# Autodesk Inventor assembly: Intake
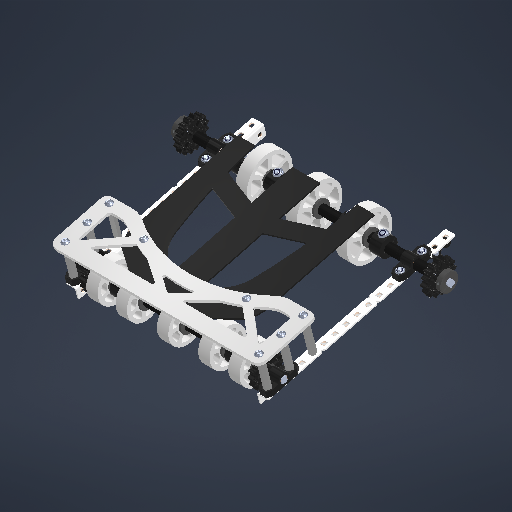
[picture p0: Inventor's stored thumbnail of the model, 512x512]
Saved by Autodesk Inventor 2025 (Build 290162000, 162)
## iProperties
Created: 2024-12-18
Part Number: Intake
Document SubType Name: Assembly
Designer: Juan
Author: Juan
## Documents named in this file (30)
- C:\Users\Juan\Documents\GitHub\ATUM-VRC-High-Stakes-CAD\Robot\Subassemblies\Intake.iam
- C:\Users\Juan\Documents\GitHub\ATUM-VRC-High-Stakes-CAD\VEX-CAD-Inventor\Motion\Shaft HS\Shaft HS\Shaft HS 9.0 in.ipt
- C:\Users\Juan\Documents\GitHub\ATUM-VRC-High-Stakes-CAD\VEX-CAD-Inventor\Motion\Shaft HS\Shaft HS.ipt
- C:\Users\Juan\Documents\GitHub\ATUM-VRC-High-Stakes-CAD\VEX-CAD-Inventor\Structure\Angle\Aluminum 1x1\Alu Angle 1x1x17.ipt
- C:\Users\Juan\Documents\GitHub\ATUM-VRC-High-Stakes-CAD\VEX-CAD-Inventor\Motion\Shaft HS\HS Pillow Bearing Block.ipt
- C:\Users\Juan\Documents\GitHub\ATUM-VRC-High-Stakes-CAD\VEX-CAD-Inventor\Motion\Sprockets\6P Sprocket\6P 16T Sprocket, No Insert.iam
- C:\Users\Juan\Documents\GitHub\ATUM-VRC-High-Stakes-CAD\VEX-CAD-Inventor\Motion\Sprockets\6P Sprocket.iam
- C:\Users\Juan\Documents\GitHub\ATUM-VRC-High-Stakes-CAD\VEX-CAD-Inventor\Structure\Hardware\Screw Steel - Star\SScrew Star Threaded .375.ipt
- C:\Users\Juan\Documents\GitHub\ATUM-VRC-High-Stakes-CAD\VEX-CAD-Inventor\Structure\Hardware\Screw Steel - Star.ipt
- C:\Users\Juan\Documents\GitHub\ATUM-VRC-High-Stakes-CAD\VEX-CAD-Inventor\Structure\Standoff\Standoff 1.50.ipt
- C:\Users\Juan\Documents\GitHub\ATUM-VRC-High-Stakes-CAD\VEX-CAD-Inventor\Structure\Standoff.ipt
- C:\Users\Juan\Documents\GitHub\ATUM-VRC-High-Stakes-CAD\VEX-CAD-Inventor\Motion\1-Post Bearing Flat Hex Retainer.ipt
- C:\Users\Juan\Documents\GitHub\ATUM-VRC-High-Stakes-CAD\VEX-CAD-Inventor\Motion\Shaft HS\Shaft HS\Shaft HS 12.0 in.ipt
- C:\Users\Juan\Documents\GitHub\ATUM-VRC-High-Stakes-CAD\VEX-CAD-Inventor\Motion\Shaft HS\HS Shaft Collar.ipt
- C:\Users\Juan\Documents\GitHub\ATUM-VRC-High-Stakes-CAD\VEX-CAD-Inventor\Motion\Shaft HS\HS Spacer\HSpacer .5000.ipt
- C:\Users\Juan\Documents\GitHub\ATUM-VRC-High-Stakes-CAD\VEX-CAD-Inventor\Motion\Shaft HS\HS Spacer.ipt
- C:\Users\Juan\Documents\GitHub\ATUM-VRC-High-Stakes-CAD\VEX-CAD-Inventor\Motion\Shaft HS\Low Profile HS Shaft Collar.ipt
- C:\Users\Juan\Documents\GitHub\ATUM-VRC-High-Stakes-CAD\VEX-CAD-Inventor\Motion\Shaft HS\HS Spacer\HSpacer .2500.ipt
- C:\Users\Juan\Documents\GitHub\ATUM-VRC-High-Stakes-CAD\Robot\Subassemblies\2.0 Flex Wheel with Insert.iam
- C:\Users\Juan\Documents\GitHub\ATUM-VRC-High-Stakes-CAD\VEX-CAD-Inventor\Structure\Hardware\Nut Thin Nylock.ipt
- C:\Users\Juan\Documents\GitHub\ATUM-VRC-High-Stakes-CAD\VEX-CAD-Inventor\Structure\Hardware\Screw Steel - Star\SScrew Star Smooth .625.ipt
- C:\Users\Juan\Documents\GitHub\ATUM-VRC-High-Stakes-CAD\VEX-CAD-Inventor\Motion\Shaft HS\HS Spacer\HSpacer .1250.ipt
- C:\Users\Juan\Documents\GitHub\ATUM-VRC-High-Stakes-CAD\VEX-CAD-Inventor\Motion\Shaft HS\HS Spacer\HSpacer .0625.ipt
- C:\Users\Juan\Documents\GitHub\ATUM-VRC-High-Stakes-CAD\VEX-CAD-Inventor\Structure\Hardware\Screw Steel - Star\SScrew Star Smooth .375.ipt
- C:\Users\Juan\Documents\GitHub\ATUM-VRC-High-Stakes-CAD\Robot\Subassemblies\1.625 Flex Wheel with Insert.iam
- C:\Users\Juan\Documents\GitHub\ATUM-VRC-High-Stakes-CAD\Protobot\Intake (Metal).ipt
- C:\Users\Juan\Documents\GitHub\ATUM-VRC-High-Stakes-CAD\VEX-CAD-Inventor\Motion\Spacers\Washer Steel\SWasher .375 OD x .062500.ipt
- C:\Users\Juan\Documents\GitHub\ATUM-VRC-High-Stakes-CAD\VEX-CAD-Inventor\Motion\Spacers\Washer Steel.ipt
- C:\Users\Juan\Documents\GitHub\ATUM-VRC-High-Stakes-CAD\VEX-CAD-Inventor\Motion\Spacers\Washer Steel\SWasher .375 OD x .015625.ipt
- C:\Users\Juan\Documents\GitHub\ATUM-VRC-High-Stakes-CAD\Protobot\Intake Hood.ipt
## Components (104 placed, 23 different names)
1. Shaft HS 9.0 in:1
2. Alu Angle 1x1x17:1 — Rigid:31, Rigid:37
3. HS Pillow Bearing Block:4
4. Alu Angle 1x1x17:2 — Rigid:32, Rigid:56
5. HS Pillow Bearing Block:1
6. HS Pillow Bearing Block:2
7. 6P 16T Sprocket, No Insert:1 [sub-assembly]
8. 6P 16T Sprocket, No Insert:2 [sub-assembly]
9. SScrew Star Threaded .375:1
10. Standoff 1.50:1 — Mate:120, Mate:122
11. Standoff 1.50:2 — Mate:121
12. Standoff 1.50:3
13. Standoff 1.50:4
14. 1-Post Bearing Flat Hex Retainer:1
15. HS Pillow Bearing Block:3
16. Shaft HS 12.0 in:2
17. 6P 16T Sprocket, No Insert:3 [sub-assembly]
18. 6P 16T Sprocket, No Insert:4 [sub-assembly]
19. HS Shaft Collar:1
20. HS Shaft Collar:2
21. HSpacer .5000:1
22. HSpacer .5000:2
23. HSpacer .5000:3
24. HSpacer .5000:4
25. Low Profile HS Shaft Collar:1
26. Low Profile HS Shaft Collar:2
27. HS Shaft Collar:3
28. HS Shaft Collar:4
29. HSpacer .2500:5
30. HSpacer .2500:6
31. 2.0 Flex Wheel with Insert:1 [sub-assembly]
32. 1-Post Bearing Flat Hex Retainer:2
33. 2.0 Flex Wheel with Insert:2 [sub-assembly]
34. 2.0 Flex Wheel with Insert:3 [sub-assembly]
35. HSpacer .5000:7
36. Nut Thin Nylock:1
37. HSpacer .5000:8
38. SScrew Star Smooth .625:2
39. SScrew Star Smooth .625:3
40. SScrew Star Smooth .625:4
41. SScrew Star Smooth .625:5
42. Nut Thin Nylock:2
43. Nut Thin Nylock:3
44. Nut Thin Nylock:4
45. HSpacer .5000:9
46. HSpacer .5000:10
47. HSpacer .1250:11
48. HSpacer .1250:12
49. HSpacer .0625:13
50. HSpacer .1250:14
51. HSpacer .1250:15
52. HSpacer .0625:16
53. HSpacer .0625:17
54. Nut Thin Nylock:5
55. Nut Thin Nylock:6
56. Nut Thin Nylock:7
57. Nut Thin Nylock:8
58. SScrew Star Smooth .375:6
59. SScrew Star Smooth .375:7
60. SScrew Star Smooth .375:8
61. SScrew Star Smooth .375:9
62. SScrew Star Smooth .375:14
63. SScrew Star Smooth .375:15
64. SScrew Star Smooth .375:16
65. SScrew Star Smooth .375:17
66. 1.625 Flex Wheel with Insert:1 [sub-assembly]
67. 1.625 Flex Wheel with Insert:2 [sub-assembly]
68. 1.625 Flex Wheel with Insert:3 [sub-assembly]
69. 1.625 Flex Wheel with Insert:4 [sub-assembly]
70. 1.625 Flex Wheel with Insert:5 [sub-assembly]
71. HSpacer .5000:18
72. HSpacer .1250:19
73. HSpacer .1250:20
74. HSpacer .5000:21
75. HSpacer .5000:22
76. HSpacer .5000:23
77. HS Shaft Collar:5
78. Nut Thin Nylock:9
79. SScrew Star Smooth .625:18
80. HS Shaft Collar:6
81. Nut Thin Nylock:10
82. SScrew Star Smooth .625:19
83. HSpacer .1250:24
84. HSpacer .1250:25
85. Intake (Metal):1 — Mate:120, Mate:121, Mate:122, Rigid:38, Rigid:39, Rigid:40, Rigid:41, Rigid:42, Rigid:43, Mate:125, Rigid:44, Rigid:48, Mate:126
86. Standoff 1.50:5 — Rigid:32, Rigid:36
87. Standoff 1.50:6 — Rigid:31, Rigid:33
88. SWasher .375 OD x .062500:1 — Rigid:33, Rigid:34
89. SWasher .375 OD x .015625:3 — Rigid:34
90. SWasher .375 OD x .062500:5 — Rigid:36
91. SWasher .375 OD x .015625:6
92. SScrew Star Smooth .375:20 — Rigid:39
93. SScrew Star Smooth .375:21 — Rigid:38
94. SScrew Star Smooth .375:22 — Rigid:37
95. SScrew Star Smooth .375:23 — Rigid:40
96. SScrew Star Smooth .375:24 — Rigid:43
97. SScrew Star Smooth .375:25 — Rigid:42
98. SScrew Star Smooth .375:26 — Rigid:41
99. Intake Hood:1 — Mate:125, Rigid:50, Mate:126, Mate:127
100. SScrew Star Smooth .375:29 — Rigid:48, Mate:127
101. SScrew Star Smooth .375:32 — Rigid:44
102. Nut Thin Nylock:12 — Rigid:50
103. Nut Thin Nylock:17
104. SScrew Star Smooth .375:33 — Rigid:56
## Relationships (175: Mate 121, WeldJoint 43, CylindricalJoint 9, Flush 1, Angle 1)
- [Mate]: Alu Angle 1x1x17:1 ↔ HS Pillow Bearing Block:1
- [Mate]: Alu Angle 1x1x17:1 ↔ HS Pillow Bearing Block:1
- [Mate]: Alu Angle 1x1x17:1 ↔ HS Pillow Bearing Block:1
- [Mate]: Shaft HS 9.0 in:1 ↔ HS Pillow Bearing Block:1
- [Mate]: Alu Angle 1x1x17:2 ↔ HS Pillow Bearing Block:2
- [Mate]: Alu Angle 1x1x17:2 ↔ HS Pillow Bearing Block:2
- [Mate]: Alu Angle 1x1x17:2 ↔ HS Pillow Bearing Block:2
- [Mate]: Shaft HS 9.0 in:1 ↔ HS Pillow Bearing Block:2
- [Mate]: Shaft HS 9.0 in:1 ↔ 6P 16T Sprocket, No Insert:2
- [Mate]: Shaft HS 9.0 in:1 ↔ 6P 16T Sprocket, No Insert:1
- [Mate]: Alu Angle 1x1x17:1 ↔ SScrew Star Threaded .375:1
- [Mate]: Alu Angle 1x1x17:1 ↔ 6P 16T Sprocket, No Insert:2
- [Mate]: Alu Angle 1x1x17:1 ↔ SScrew Star Threaded .375:1
- [Mate]: Alu Angle 1x1x17:1 ↔ Alu Angle 1x1x17:2
- [Mate]: HS Pillow Bearing Block:1 ↔ Standoff 1.50:1
- [Mate]: HS Pillow Bearing Block:1 ↔ Standoff 1.50:2
- [Mate]: HS Pillow Bearing Block:1 ↔ Standoff 1.50:1
- [Mate]: HS Pillow Bearing Block:1 ↔ Standoff 1.50:2
- [Mate]: HS Pillow Bearing Block:2 ↔ Standoff 1.50:4
- [Mate]: HS Pillow Bearing Block:2 ↔ Standoff 1.50:3
- [Mate]: HS Pillow Bearing Block:2 ↔ Standoff 1.50:4
- [Mate]: HS Pillow Bearing Block:2 ↔ Standoff 1.50:3
- [Mate]: Alu Angle 1x1x17:2 ↔ HS Pillow Bearing Block:3
- [Mate]: Alu Angle 1x1x17:2 ↔ HS Pillow Bearing Block:3
- [Mate]: Alu Angle 1x1x17:2 ↔ HS Pillow Bearing Block:3
- [Mate]: Shaft HS 12.0 in:2 ↔ 6P 16T Sprocket, No Insert:3
- [Mate]: Shaft HS 12.0 in:2 ↔ 6P 16T Sprocket, No Insert:4
- [Mate]: Shaft HS 12.0 in:2 ↔ 2.0 Flex Wheel with Insert:3
- [Mate]: Shaft HS 12.0 in:2 ↔ 2.0 Flex Wheel with Insert:2
- [Mate]: Shaft HS 12.0 in:2 ↔ 2.0 Flex Wheel with Insert:1
- [Mate]: Shaft HS 12.0 in:2 ↔ HSpacer .5000:4
- [Mate]: Shaft HS 12.0 in:2 ↔ HSpacer .5000:4
- [Mate]: Shaft HS 12.0 in:2 ↔ HS Shaft Collar:1
- [Mate]: Shaft HS 12.0 in:2 ↔ HS Shaft Collar:1
- [Mate]: Shaft HS 12.0 in:2 ↔ HSpacer .5000:1
- [Mate]: Shaft HS 12.0 in:2 ↔ HSpacer .5000:1
- [Mate]: HSpacer .5000:1 ↔ HSpacer .5000:4
- [Mate]: HS Shaft Collar:1 ↔ HSpacer .5000:4
- [Mate]: HS Shaft Collar:1 ↔ 2.0 Flex Wheel with Insert:3
- [Mate]: HSpacer .5000:1 ↔ 2.0 Flex Wheel with Insert:2
- [Mate]: Shaft HS 12.0 in:2 ↔ HS Shaft Collar:2
- [Mate]: Shaft HS 12.0 in:2 ↔ HS Shaft Collar:2
- [Mate]: Shaft HS 12.0 in:2 ↔ HSpacer .5000:3
- [Mate]: Shaft HS 12.0 in:2 ↔ HSpacer .5000:3
- [Mate]: Shaft HS 12.0 in:2 ↔ HSpacer .5000:2
- [Mate]: Shaft HS 12.0 in:2 ↔ HSpacer .5000:2
- [Mate]: HSpacer .5000:2 ↔ 2.0 Flex Wheel with Insert:2
- [Mate]: HSpacer .5000:2 ↔ HSpacer .5000:3
- [Mate]: HS Shaft Collar:2 ↔ HSpacer .5000:3
- [Mate]: HS Shaft Collar:2 ↔ 2.0 Flex Wheel with Insert:1
- [Mate] (36.1696 mm): Alu Angle 1x1x17:1 ↔ 2.0 Flex Wheel with Insert:3
- [Mate]: Shaft HS 12.0 in:2 ↔ Low Profile HS Shaft Collar:2
- [Mate]: Shaft HS 12.0 in:2 ↔ Low Profile HS Shaft Collar:2
- [Mate]: 6P 16T Sprocket, No Insert:3 ↔ Low Profile HS Shaft Collar:2
- [Mate]: Shaft HS 12.0 in:2 ↔ Low Profile HS Shaft Collar:1
- [Mate]: Shaft HS 12.0 in:2 ↔ Low Profile HS Shaft Collar:1
- [Mate]: 6P 16T Sprocket, No Insert:4 ↔ Low Profile HS Shaft Collar:1
- [Mate]: Shaft HS 12.0 in:2 ↔ HS Shaft Collar:3
- [Mate]: Shaft HS 12.0 in:2 ↔ HS Shaft Collar:3
- [Mate]: Shaft HS 12.0 in:2 ↔ HS Shaft Collar:4
- [Mate]: Shaft HS 12.0 in:2 ↔ HS Shaft Collar:4
- [Mate]: Shaft HS 12.0 in:2 ↔ HSpacer .2500:5
- [Mate]: Shaft HS 12.0 in:2 ↔ HSpacer .2500:5
- [Mate]: Shaft HS 12.0 in:2 ↔ HSpacer .2500:6
- [Mate]: Shaft HS 12.0 in:2 ↔ HSpacer .2500:6
- [Mate]: HSpacer .2500:6 ↔ 2.0 Flex Wheel with Insert:3
- [Mate]: HSpacer .2500:5 ↔ 2.0 Flex Wheel with Insert:1
- [Mate]: HS Shaft Collar:4 ↔ HSpacer .2500:5
- [Mate]: HS Shaft Collar:3 ↔ HSpacer .2500:6
- [WeldJoint]: HS Shaft Collar:3 ↔ SScrew Star Smooth .625:2
- [WeldJoint]: HS Shaft Collar:1 ↔ SScrew Star Smooth .625:5
- [WeldJoint]: HS Shaft Collar:2 ↔ SScrew Star Smooth .625:4
- [WeldJoint]: HS Shaft Collar:4 ↔ SScrew Star Smooth .625:3
- [WeldJoint]: HS Shaft Collar:3 ↔ Nut Thin Nylock:1
- [WeldJoint]: HS Shaft Collar:4 ↔ Nut Thin Nylock:2
- [WeldJoint]: HS Shaft Collar:2 ↔ Nut Thin Nylock:3
- [WeldJoint]: HS Shaft Collar:1 ↔ Nut Thin Nylock:4
- [WeldJoint]: HS Shaft Collar:3 ↔ HSpacer .5000:7
- [WeldJoint]: HS Shaft Collar:4 ↔ HSpacer .5000:9
- [Mate]: Shaft HS 12.0 in:2 ↔ HSpacer .5000:8
- [Mate]: 6P 16T Sprocket, No Insert:3 ↔ HSpacer .5000:8
- [Mate]: Shaft HS 12.0 in:2 ↔ HSpacer .5000:10
- [Mate]: 6P 16T Sprocket, No Insert:4 ↔ HSpacer .5000:10
- [Mate]: Shaft HS 12.0 in:2 ↔ HSpacer .1250:12
- [Mate]: HSpacer .5000:10 ↔ HSpacer .1250:12
- [Mate]: HSpacer .5000:9 ↔ HSpacer .1250:11
- [Mate]: HSpacer .5000:9 ↔ HSpacer .1250:11
- [Mate]: HSpacer .1250:11 ↔ HSpacer .0625:13
- [Mate]: HSpacer .1250:11 ↔ HSpacer .0625:13
- [Mate]: HSpacer .5000:8 ↔ HSpacer .1250:14
- [Mate]: HSpacer .5000:8 ↔ HSpacer .1250:14
- [Mate]: HSpacer .1250:14 ↔ HSpacer .0625:16
- [Mate]: HSpacer .1250:14 ↔ HSpacer .0625:16
- [Mate]: HSpacer .5000:7 ↔ HSpacer .1250:15
- [Mate]: HSpacer .5000:7 ↔ HSpacer .1250:15
- [Mate]: HSpacer .1250:15 ↔ HSpacer .0625:17
- [Mate]: HSpacer .1250:15 ↔ HSpacer .0625:17
- [WeldJoint]: HS Pillow Bearing Block:3 ↔ Nut Thin Nylock:7
- [WeldJoint]: HS Pillow Bearing Block:3 ↔ Nut Thin Nylock:8
- [WeldJoint]: Alu Angle 1x1x17:1 ↔ SScrew Star Smooth .375:6
- [WeldJoint]: Alu Angle 1x1x17:1 ↔ SScrew Star Smooth .375:7
- [WeldJoint]: Alu Angle 1x1x17:2 ↔ SScrew Star Smooth .375:9
- [WeldJoint]: Alu Angle 1x1x17:2 ↔ SScrew Star Smooth .375:8
- [WeldJoint]: Alu Angle 1x1x17:2 ↔ SScrew Star Smooth .375:15
- [WeldJoint]: Alu Angle 1x1x17:2 ↔ SScrew Star Smooth .375:14
- [WeldJoint]: Alu Angle 1x1x17:1 ↔ SScrew Star Smooth .375:17
- [WeldJoint]: Alu Angle 1x1x17:1 ↔ SScrew Star Smooth .375:16
- [CylindricalJoint]: Shaft HS 9.0 in:1 ↔ 1.625 Flex Wheel with Insert:1
- [CylindricalJoint]: Shaft HS 9.0 in:1 ↔ 1.625 Flex Wheel with Insert:5
- [Mate]: 1.625 Flex Wheel with Insert:5 ↔ HSpacer .5000:18
- [Mate]: 1.625 Flex Wheel with Insert:5 ↔ HSpacer .1250:19
- [Mate]: 1.625 Flex Wheel with Insert:5 ↔ HSpacer .1250:19
- [Mate]: HSpacer .5000:18 ↔ HSpacer .1250:19
- [Mate]: 1.625 Flex Wheel with Insert:5 ↔ HSpacer .1250:20
- [Mate]: 1.625 Flex Wheel with Insert:5 ↔ HSpacer .1250:20
- [Mate]: 1.625 Flex Wheel with Insert:5 ↔ HSpacer .5000:21
- [Mate]: HSpacer .1250:20 ↔ HSpacer .5000:21
- [Mate]: 1.625 Flex Wheel with Insert:5 ↔ HSpacer .5000:23
- [Mate]: HSpacer .5000:18 ↔ HSpacer .5000:23
- [Mate]: 1.625 Flex Wheel with Insert:5 ↔ HSpacer .5000:22
- [Mate]: HSpacer .5000:21 ↔ HSpacer .5000:22
- [Mate]: 1.625 Flex Wheel with Insert:1 ↔ HSpacer .5000:23
- [CylindricalJoint]: Shaft HS 9.0 in:1 ↔ 1.625 Flex Wheel with Insert:4
- [Mate]: 1.625 Flex Wheel with Insert:4 ↔ HSpacer .5000:22
- [CylindricalJoint]: Shaft HS 9.0 in:1 ↔ 1.625 Flex Wheel with Insert:3
- [CylindricalJoint]: Shaft HS 9.0 in:1 ↔ 1.625 Flex Wheel with Insert:2
- [WeldJoint]: HS Shaft Collar:5 ↔ SScrew Star Smooth .625:18
- [WeldJoint]: HS Shaft Collar:5 ↔ Nut Thin Nylock:9
- [WeldJoint]: HS Shaft Collar:6 ↔ SScrew Star Smooth .625:19
- [WeldJoint]: HS Shaft Collar:6 ↔ Nut Thin Nylock:10
- [CylindricalJoint]: Shaft HS 9.0 in:1 ↔ HS Shaft Collar:5
- [CylindricalJoint]: Shaft HS 9.0 in:1 ↔ HS Shaft Collar:6
- [Mate]: 6P 16T Sprocket, No Insert:1 ↔ 1.625 Flex Wheel with Insert:2
- [Mate]: 1.625 Flex Wheel with Insert:2 ↔ HS Shaft Collar:6
- [Mate]: 6P 16T Sprocket, No Insert:2 ↔ 1.625 Flex Wheel with Insert:3
- [Mate]: 1.625 Flex Wheel with Insert:3 ↔ HS Shaft Collar:5
- [Mate]: Alu Angle 1x1x17:2 ↔ 6P 16T Sprocket, No Insert:1
- [Flush]: HS Shaft Collar:5 ↔ HS Shaft Collar:6
- [Angle] (0 deg): Shaft HS 9.0 in:1 ↔ HS Shaft Collar:5
- [CylindricalJoint]: Shaft HS 9.0 in:1 ↔ HSpacer .1250:25
- [Mate]: HS Shaft Collar:5 ↔ HSpacer .1250:25
- [Mate]: 1.625 Flex Wheel with Insert:1 ↔ HSpacer .1250:25
- [CylindricalJoint]: Shaft HS 9.0 in:1 ↔ HSpacer .1250:24
- [Mate]: 1.625 Flex Wheel with Insert:4 ↔ HSpacer .1250:24
- [Mate]: Alu Angle 1x1x17:1 ↔ HS Pillow Bearing Block:4
- [Mate]: Alu Angle 1x1x17:1 ↔ HS Pillow Bearing Block:4
- [Mate]: Alu Angle 1x1x17:1 ↔ HS Pillow Bearing Block:4
- [Mate]: HS Pillow Bearing Block:4 ↔ Shaft HS 12.0 in:2
- [WeldJoint]: HS Pillow Bearing Block:4 ↔ Nut Thin Nylock:6
- [WeldJoint]: HS Pillow Bearing Block:4 ↔ Nut Thin Nylock:5
- [Mate]: Alu Angle 1x1x17:1 ↔ 1-Post Bearing Flat Hex Retainer:2
- [Mate]: SScrew Star Threaded .375:1 ↔ 1-Post Bearing Flat Hex Retainer:2
- Mate:120: Standoff 1.50:1 ↔ Intake (Metal):1
- Mate:121: Standoff 1.50:2 ↔ Intake (Metal):1
- Mate:122: Standoff 1.50:1 ↔ Intake (Metal):1
- Rigid:31 [WeldJoint]: Alu Angle 1x1x17:1 ↔ Standoff 1.50:6
- Rigid:32 [WeldJoint]: Alu Angle 1x1x17:2 ↔ Standoff 1.50:5
- Rigid:33 [WeldJoint]: Standoff 1.50:6 ↔ SWasher .375 OD x .062500:1
- Rigid:34 [WeldJoint]: SWasher .375 OD x .062500:1 ↔ SWasher .375 OD x .015625:3
- [WeldJoint]: SWasher .375 OD x .062500:5 ↔ SWasher .375 OD x .015625:6
- Rigid:36 [WeldJoint]: Standoff 1.50:5 ↔ SWasher .375 OD x .062500:5
- Rigid:37 [WeldJoint]: Alu Angle 1x1x17:1 ↔ SScrew Star Smooth .375:22
- Rigid:38 [WeldJoint]: Intake (Metal):1 ↔ SScrew Star Smooth .375:21
- Rigid:39 [WeldJoint]: Intake (Metal):1 ↔ SScrew Star Smooth .375:20
- Rigid:40 [WeldJoint]: Intake (Metal):1 ↔ SScrew Star Smooth .375:23
- Rigid:41 [WeldJoint]: Intake (Metal):1 ↔ SScrew Star Smooth .375:26
- Rigid:42 [WeldJoint]: Intake (Metal):1 ↔ SScrew Star Smooth .375:25
- Rigid:43 [WeldJoint]: Intake (Metal):1 ↔ SScrew Star Smooth .375:24
- Mate:125: Intake (Metal):1 ↔ Intake Hood:1
- Rigid:44 [WeldJoint]: Intake (Metal):1 ↔ SScrew Star Smooth .375:32
- Rigid:48 [WeldJoint]: Intake (Metal):1 ↔ SScrew Star Smooth .375:29
- Rigid:50 [WeldJoint]: Intake Hood:1 ↔ Nut Thin Nylock:12
- Rigid:56 [WeldJoint]: Alu Angle 1x1x17:2 ↔ SScrew Star Smooth .375:33
- Mate:126: Intake (Metal):1 ↔ Intake Hood:1
- Mate:127: Intake Hood:1 ↔ SScrew Star Smooth .375:29
## Named parameters: d2183_d2114 = 0 mm, d2184_d2118 = 0 mm, d2185_d2183_d2114 = 0 mm, d2186_d2184_d2118 = 0 mm, d178_d177 = 0 mm
